# Autodesk Inventor assembly: y_plate_assembly
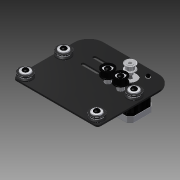
[picture p0: Inventor's stored thumbnail of the model, 180x180]
Saved by Autodesk Inventor 2014 (Build 180170000, 170)
## iProperties
Created: 2013-07-17
Part Number: y_plate_assembly
Document SubType Name: Assembly
Designer: Edward
Author: Edward
## Documents named in this file (14)
- C:\Users\Edward\Desktop\Shapeoko_v2.0\shapeoko_lowpro\y_plate_assembly.iam
- C:\Users\Edward\Desktop\Shapeoko_v2.0\motor_mount_v2.ipt
- C:\Users\Edward\Desktop\Shapeoko_v2.0\B18033.ipt
- C:\Users\Edward\Desktop\Shapeoko_v2.0\B30037.iam
- C:\Users\Edward\Desktop\Shapeoko_v2.0\SM-H03.ipt
- C:\Users\Edward\Desktop\Shapeoko_v2.0\91239A233.ipt
- C:\Users\Edward\Desktop\Shapeoko_v2.0\SM-H04.ipt
- C:\Users\Edward\Downloads\M1173041- NEMA 17.ipt
- C:\Users\Edward\Desktop\Shapeoko_v2.0\B30041.iam
- C:\Users\Edward\Desktop\Shapeoko_v2.0\91239A236.ipt
- C:\Users\Edward\Desktop\Shapeoko_v2.0\AS38-12-20.ipt
- C:\Users\Edward\Desktop\Shapeoko_v2.0\a_6a51-020df0606.ipt
- C:\Users\Edward\Desktop\Shapeoko_v2.0\91290A113.ipt
- C:\Users\Edward\Desktop\Shapeoko_v2.0\91166A210.ipt
## Components (41 placed, 13 different names)
1. motor_mount_v2:1 — Insert:10, Mate:3, Insert:11, Insert:12, Insert:18, Mate:5, Insert:19, Insert:20, Insert:21, Insert:25, Insert:27, Angle:1, Insert:34, Insert:38, Insert:39, Insert:40
2. B18033:1 — Insert:10
3. B30037:1 [sub-assembly]
4. SM-H03:1 — Insert:11
5. 91239A233:1
6. SM-H04:1
7. SM-H03:2 — Mate:3
8. SM-H03:3 — Insert:12
9. 91239A233:2
10. B30037:2 [sub-assembly]
11. B18033:2 — Insert:18
12. B30037:3 [sub-assembly]
13. SM-H03:4 — Insert:20
14. 91239A233:3
15. SM-H04:2
16. SM-H03:5 — Mate:5
17. SM-H03:6 — Insert:19
18. 91239A233:4
19. B30037:4 [sub-assembly]
20. M1173041- NEMA 17:1 — Insert:21, Mate:6, Angle:1, Insert:32
21. a_6a51-020df0606:1 — Mate:6, Insert:32
22. 91290A113:1
23. 91166A210:1 — Insert:34
24. 91290A113:2
25. 91166A210:2 — Insert:38
26. 91290A113:3
27. 91166A210:3 — Insert:39
28. 91290A113:4
29. 91166A210:4 — Insert:40
30. 91239A236:1
31. B30041:1 [sub-assembly]
32. AS38-12-20:1
33. SM-H03:7 — Insert:25
34. SM-H03:8 — Insert:27
35. SM-H04:4
36. 91239A236:2
37. B30041:2 [sub-assembly]
38. AS38-12-20:2
39. SM-H03:9
40. SM-H03:10
41. SM-H04:5
## Component patterns: (2 elements, first: 91239A236:1 + B30041:1 + AS38-12-20:1 + SM-H03:7 + SM-H03:8 + SM-H04:4)
## Relationships (38: Insert 32, Mate 5, Angle 1)
- [Insert]: B30037:1 ↔ SM-H03:1
- [Insert]: B30037:1 ↔ 91239A233:1
- [Insert]: SM-H04:1 ↔ SM-H03:3
- [Insert]: SM-H03:2 ↔ B30037:2
- [Insert]: 91239A233:2 ↔ B30037:2
- [Mate]: B18033:1 ↔ 91239A233:2
- Insert:10: motor_mount_v2:1 ↔ B18033:1
- Mate:3: motor_mount_v2:1 ↔ SM-H03:2
- Insert:11: motor_mount_v2:1 ↔ SM-H03:1
- Insert:12: motor_mount_v2:1 ↔ SM-H03:3
- [Insert]: B30037:3 ↔ SM-H03:4
- [Insert]: B30037:3 ↔ 91239A233:3
- [Insert]: SM-H04:2 ↔ SM-H03:6
- [Insert]: SM-H03:5 ↔ B30037:4
- [Insert]: 91239A233:4 ↔ B30037:4
- [Mate]: B18033:2 ↔ 91239A233:4
- Insert:18: motor_mount_v2:1 ↔ B18033:2
- Mate:5: motor_mount_v2:1 ↔ SM-H03:5
- Insert:19: motor_mount_v2:1 ↔ SM-H03:6
- Insert:20: motor_mount_v2:1 ↔ SM-H03:4
- Insert:21: motor_mount_v2:1 ↔ M1173041- NEMA 17:1
- [Insert]: 91239A236:1 ↔ B30041:1
- [Insert]: B30041:1 ↔ AS38-12-20:1
- [Insert]: AS38-12-20:1 ↔ SM-H03:7
- Insert:25: motor_mount_v2:1 ↔ SM-H03:7
- Mate:6: M1173041- NEMA 17:1 ↔ a_6a51-020df0606:1
- [Insert]: SM-H03:8 ↔ SM-H04:4
- Insert:27: motor_mount_v2:1 ↔ SM-H03:8
- Angle:1 (0 deg): motor_mount_v2:1 ↔ M1173041- NEMA 17:1
- Insert:32: M1173041- NEMA 17:1 ↔ a_6a51-020df0606:1
- [Insert]: 91290A113:1 ↔ 91166A210:1
- Insert:34: motor_mount_v2:1 ↔ 91166A210:1
- [Insert]: 91290A113:2 ↔ 91166A210:2
- [Insert]: 91290A113:3 ↔ 91166A210:3
- [Insert]: 91290A113:4 ↔ 91166A210:4
- Insert:38: motor_mount_v2:1 ↔ 91166A210:2
- Insert:39: motor_mount_v2:1 ↔ 91166A210:3
- Insert:40: motor_mount_v2:1 ↔ 91166A210:4
## Named parameters: d6_d1 = 0 mm, d8_d9 = 0 mm, d9_d10 = 0 mm, d10_d11 = 0 mm, d17_d1 = 0 mm, d18_d7 = 0 mm, d22_d12 = 0 mm, d36_d9 = 0 mm, d182_d39 = 0 mm, d51_d182_d39 = 0 mm, d52_d182_d39 = 0 mm, d53_d182_d39 = 0 mm
